# Autodesk Inventor assembly: main_assembly
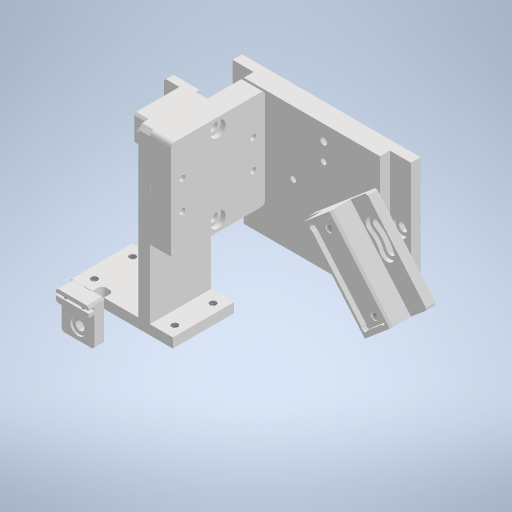
[picture p0: Inventor's stored thumbnail of the model, 512x512]
Saved by Autodesk Inventor 2024.2 (Build 282272000, 272)
## iProperties
Created: 2024-02-21
Part Number: main_assembly
Document SubType Name: Assembly
Designer: fabig
Author: fabig
## Documents named in this file (3)
- C:\Users\fabig\OneDrive\Documents\GitHub\Git Scheme testing\Parent-folder-table-assembly-\main_assembly.iam
- C:\Users\fabig\OneDrive\Documents\GitHub\Git Scheme testing\Parent-folder-table-assembly-\Subproject assemblies\project1-assembly\project1-assembly.iam
- C:\Users\fabig\OneDrive\Documents\GitHub\Git Scheme testing\Parent-folder-table-assembly-\Subproject assemblies\project2-assembly\project2_assembly.iam
## Components (2 placed, 2 different names)
1. project1-assembly:1 [sub-assembly] — Flush:1, Flush:2, Flush:3, Mate:1, Flush:4, Flush:5
2. project2_assembly:1 [sub-assembly] — Mate:1, Flush:4, Flush:5
## Relationships (6: Flush 5, Mate 1)
- Flush:1: project1-assembly:1
- Flush:2: project1-assembly:1
- Flush:3: project1-assembly:1
- Mate:1: project1-assembly:1 ↔ project2_assembly:1
- Flush:4: project1-assembly:1 ↔ project2_assembly:1
- Flush:5: project1-assembly:1 ↔ project2_assembly:1
